# Autodesk Inventor assembly: ImprintSample
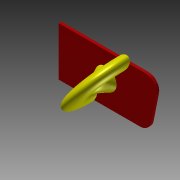
[picture p0: Inventor's stored thumbnail of the model, 180x180]
Saved by Autodesk Inventor 2014 Beta1 (Build 180079000, 79) ContinuousBuild 0
## iProperties
Created: 2012-10-22
Part Number: ImprintSample
Document SubType Name: Assembly
Designer: ekinsb
Author: ekinsb
## Documents named in this file (3)
- C:\Users\ekinsb\Documents\Presentations\AU 2012\Inventor 2014\ImprintSample.iam
- C:\Users\ekinsb\Documents\Presentations\AU 2012\Inventor 2014\ImprintPart1.ipt
- C:\Users\ekinsb\Documents\Presentations\AU 2012\Inventor 2014\ImprintPart2.ipt
## Components (2 placed, 2 different names)
1. ImprintPart1:1 — Mate:1
2. ImprintPart2:1 — Mate:1
## Relationships (1: Mate 1)
- Mate:1: ImprintPart1:1 ↔ ImprintPart2:1
